# Autodesk Inventor assembly: VerticalJagTower
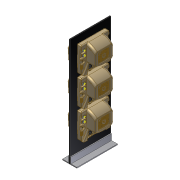
[picture p0: Inventor's stored thumbnail of the model, 180x180]
Saved by Autodesk Inventor 2012 (Build 160160000, 160)
## iProperties
Created: 2012-01-22
Part Number: VerticalJagTower
Document SubType Name: Assembly
Designer: JesseK
Mass: 13055.3 g
Surface Area: 5575.77 cm^2
Volume: 2052.37 cm^3
Density: 6.36108 g/cm^3
Author: JesseK
## Documents named in this file (4)
- Z:\UserData\Documents\Inventor\team1885frc\Robot2012\Electronics Board\VerticalJagTower.iam
- Z:\UserData\Documents\Inventor\team1885frc\Robot2012\Electronics Board\VerticalJagTower.ipt
- Z:\UserData\Documents\Inventor\team1885frc\Electronics\Jag\Jag.iam
- Z:\UserData\Documents\Inventor\team1885frc\Robot2012\Electronics Board\VerticalJagTowerMount.ipt
## Components (9 placed, 3 different names)
1. VerticalJagTower:1 — Mate:3, Mate:4, Mate:5, Mate:7, Mate:9, Mate:10, Mate:25, Mate:26, Flush:6, Flush:7, Mate:27, Mate:28
2. Jag:2 [sub-assembly] — Mate:7, Mate:15, Mate:16
3. Jag:4 [sub-assembly] — Mate:9, Mate:17, Mate:18
4. Jag:5 [sub-assembly] — Mate:10, Mate:19, Mate:20
5. Jag:8 [sub-assembly] — Mate:3, Mate:15, Mate:16, Flush:4, Mate:23
6. Jag:9 [sub-assembly] — Mate:4, Mate:17, Mate:18, Flush:4, Flush:5, Mate:23, Mate:24
7. Jag:10 [sub-assembly] — Mate:5, Mate:19, Mate:20, Flush:5, Mate:24
8. VerticalJagTowerMount:1 — Mate:26, Flush:6, Mate:28
9. VerticalJagTowerMount:2 — Mate:25, Flush:7, Mate:27
## Relationships (22: Mate 18, Flush 4)
- Mate:3: VerticalJagTower:1 ↔ Jag:8
- Mate:4: VerticalJagTower:1 ↔ Jag:9
- Mate:5: VerticalJagTower:1 ↔ Jag:10
- Mate:7: VerticalJagTower:1 ↔ Jag:2
- Mate:9: VerticalJagTower:1 ↔ Jag:4
- Mate:10: VerticalJagTower:1 ↔ Jag:5
- Mate:15: Jag:2 ↔ Jag:8
- Mate:16: Jag:2 ↔ Jag:8
- Mate:17: Jag:4 ↔ Jag:9
- Mate:18: Jag:4 ↔ Jag:9
- Mate:19: Jag:5 ↔ Jag:10
- Mate:20: Jag:5 ↔ Jag:10
- Flush:4 (107.95 mm): Jag:8 ↔ Jag:9
- Flush:5 (107.95 mm): Jag:9 ↔ Jag:10
- Mate:23: Jag:8 ↔ Jag:9
- Mate:24: Jag:9 ↔ Jag:10
- Mate:25: VerticalJagTower:1 ↔ VerticalJagTowerMount:2
- Mate:26: VerticalJagTower:1 ↔ VerticalJagTowerMount:1
- Flush:6: VerticalJagTower:1 ↔ VerticalJagTowerMount:1
- Flush:7: VerticalJagTower:1 ↔ VerticalJagTowerMount:2
- Mate:27: VerticalJagTower:1 ↔ VerticalJagTowerMount:2
- Mate:28: VerticalJagTower:1 ↔ VerticalJagTowerMount:1
